# Autodesk Inventor assembly: Complete front top housing
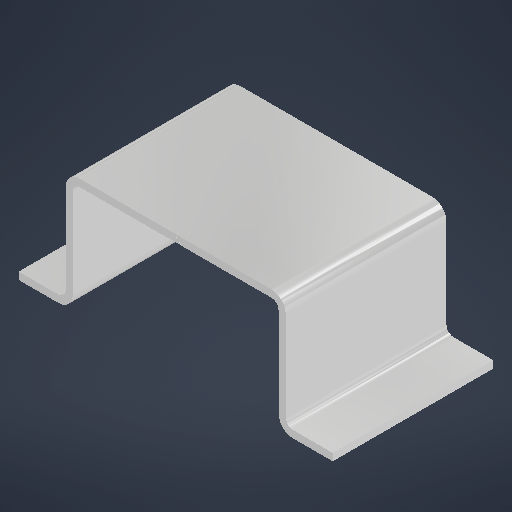
[picture p0: Inventor's stored thumbnail of the model, 512x512]
Saved by Autodesk Inventor 2026.3 (Build 303398000, 398)
## iProperties
Created: 2026-08-05
Part Number: Complete front top housing
Document SubType Name: Weldment
Designer: matot
Weld Material: Welded Aluminum-6061
Author: matot
## Documents named in this file (2)
- C:\Users\matot\OneDrive - Stellenbosch University\2026\MechatronicsProject478\Building the joint\Joint Assembly\Complete front top housing.iam
- C:\Users\matot\OneDrive - Stellenbosch University\2026\MechatronicsProject478\Building the joint\Joint Assembly\top front joint housing.ipt
## Components (2 placed, 1 different names)
1. top front joint housing:1 — Mate:1, Flush:1, Flush:2
2. top front joint housing:2 — Mate:1, Flush:1, Flush:2
## Relationships (3: Flush 2, Mate 1)
- Mate:1: top front joint housing:1 ↔ top front joint housing:2
- Flush:1: top front joint housing:1 ↔ top front joint housing:2
- Flush:2: top front joint housing:1 ↔ top front joint housing:2
